# Autodesk Inventor assembly: main_assy
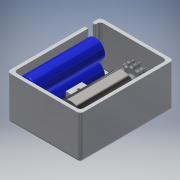
[picture p0: Inventor's stored thumbnail of the model, 180x180]
Saved by Autodesk Inventor 2017 (Build 210142000, 142)
## iProperties
Created: 2018-09-27
Part Number: main_assy
Document SubType Name: Assembly
Designer: Mitch
Author: Mitch
## Documents named in this file (5)
- E:\Youtube Channel\Pojects\Chain Blinds\Mechanical\main_assy.iam
- E:\Youtube Channel\Pojects\Chain Blinds\Mechanical\chain_gear.ipt
- E:\Youtube Channel\Pojects\Chain Blinds\Mechanical\Case Bottom.ipt
- E:\Youtube Channel\Pojects\Chain Blinds\Mechanical\battery pack.iam
- E:\Youtube Channel\Pojects\Chain Blinds\Mechanical\Motor.ipt
## Components (4 placed, 4 different names)
1. Case Bottom:1 — Tangent:1, Tangent:2, Tangent:3, Tangent:4, Tangent:5, Mate:3, Mate:4
2. battery pack:1 [sub-assembly] — Tangent:1, Tangent:2, Tangent:3, Mate:4
3. Motor:1 — Tangent:4, Mate:1, Mate:2, Tangent:5, Mate:3
4. chain_gear:1 — Mate:1, Mate:2
## Relationships (9: Tangent 5, Mate 4)
- Tangent:1: Case Bottom:1 ↔ battery pack:1
- Tangent:2: Case Bottom:1 ↔ battery pack:1
- Tangent:3: Case Bottom:1 ↔ battery pack:1
- Tangent:4 (3.175 mm): Case Bottom:1 ↔ Motor:1
- Mate:1: Motor:1 ↔ chain_gear:1
- Mate:2: Motor:1 ↔ chain_gear:1
- Tangent:5 (9.525 mm): Case Bottom:1 ↔ Motor:1
- Mate:3 (3.81 mm): Case Bottom:1 ↔ Motor:1
- Mate:4 (3.81 mm): Case Bottom:1 ↔ battery pack:1
